# Autodesk Inventor assembly: NSFMRRA10-74-B3-S3-KC31_5-A11(000_000)_MIR_CPY
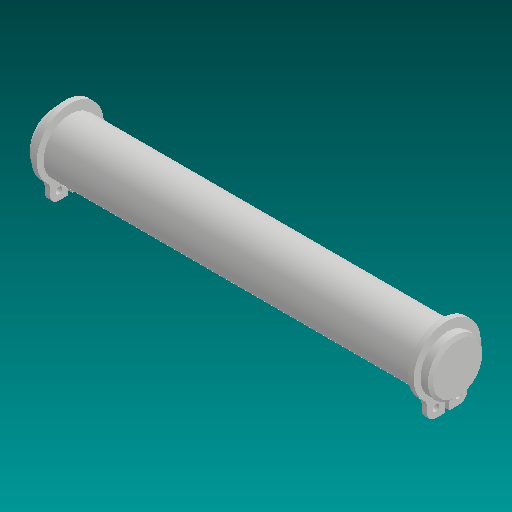
[picture p0: Inventor's stored thumbnail of the model, 512x512]
Saved by Autodesk Inventor 2020 (Build 240168000, 168)
## iProperties
Category: PARTsolutions
Company: MISUMI
Created: 2022-11-16
Part Number: NSFMRRA10-74-B3-S3-KC31_5-A11(000_000)_MIR_CPY
Catalog Web Link: www.cadenas.de
Description: NSFMRR, SFMRR, PSFMRR, SSFMRR, NSFHRR, SFHRR, PSFHRR, SSFHRR, NSFRR, SFRR, PSFRR, SSFRR, NSFMRRA, SFMRRA, PSFMRRA, SSFMRRA, NSFHRRA, SFHRRA, PSFHRRA, SSFHRRA, NSFRRA, SFRRA, PSFRRA, SSFRRA, HFRRA, PHFRRA, PSFRR PSFRRA, PSFHRR, PSFHRRA, SSFRR, SSFRRA, SSFHRR, SSFHRRA, PPSFRR, PPSFRRA, PPSFHRR, PPSFHRRA, SSSFRR, SSSFRRA, SSSFHRR, SSSFHRRA_shaft-Rotary Shafts - Retaining Ring Grooves on Both Ends - Standard
Vendor: MISUMI
Document SubType Name: Assembly
Designer: kanazawakotaro
Manufacturer: MISUMI
Mass: 5.85506 g
Surface Area: 29.329 cm^2
Volume: 5.85506 cm^3
Density: 1 g/cm^3
Title: NSFMRRA10-74-B3-S3-KC31.5-A11
Author: Cadenas PARTsolutions
Comments: Rotary Shafts - Retaining Ring Grooves on Both Ends - Standard
PSOL_IDENT_0: {$CADENAS_DATA/23d-libs/misumi/metric/11_rotary_shafts/psfrra_asmtab.prj},820 {VTYP=3D},{STYP=ASSTAB
PSOL_IDENT_1: },{NB=NSFMRRA10-74-B3-S3-KC31.5-A11(000_000)},{LINA=NSFMRRA10-74-B3-S3-KC31.5-A11},{NN=NSFMRR, SFMRR
PSOL_IDENT_2: , PSFMRR, SSFMRR, NSFHRR, SFHRR, PSFHRR, SSFHRR, NSFRR, SFRR, PSFRR, SSFRR, NSFMRRA, SFMRRA, PSFMRRA
PSOL_IDENT_3: , SSFMRRA, NSFHRRA, SFHRRA, PSFHRRA, SSFHRRA, NSFRRA, SFRRA, PSFRRA, SSFRRA, HFRRA, PHFRRA, PSFRR PS
PSOL_IDENT_4: FRRA, PSFHRR, PSFHRRA, SSFRR, SSFRRA, SSFHRR, SSFHRRA, PPSFRR, PPSFRRA, PPSFHRR, PPSFHRRA, SSSFRR, S
PSOL_IDENT_5: SSFRRA, SSSFHRR, SSSFHRRA_shaft},{DATE=21.04.2022 07:40:19},{GEOMDATE=27.07.2021 08:15:02},{VERSION=
PSOL_IDENT_6: },{LINEID=30},{WBVAR=TS,TYS,MAT,ST,ALT1,L,B,S,ALT2,KC,A,WKC,C,K,E,KZ,Z,ALT3,FC,GALT3,WFC,J,WALT3,V,A
PSOL_IDENT_7: LT4,SFC,SG,AG,ALT5,UC,ALT7,SC,ALT10,KWC,ALT11,WC,ALT32,CD,ALT34,TCJ,WTCJ,XT,HCJ,WHCJ,XH},{WBNUMERIC=
PSOL_IDENT_8: L,B,S,KC,A,WKC,C,K,E,KZ,Z,FC,GALT3,WFC,J,WALT3,V,SFC,SG,AG,UC,SC,KWC,WC,TCJ,WTCJ,XT,HCJ,WHCJ,XH}  {N
PSOL_IDENT_9: B=NSFMRRA10-74-B3-S3-KC31.5-A11(000_000)},{LINA=NSFMRRA10-74-B3-S3-KC31.5-A11},{KT=DUMMY},{PN=NSFMRR
PSOL_IDENT_10: A10-74-B3-S3-KC31.5-A11},{TYPE=NSFMRRA},{TS=SWR},{TYS=H9},{TYSALG= 'H9','h9 (Cold-drawn)','H7','h7 (
PSOL_IDENT_11: Ground)','G6','g6 (Ground)' },{MAT=S45C},{MATALG= 'S45C','S45C Equivalent', 'SUS304','SUS304' },{ST=
PSOL_IDENT_12: },{STALG= '','-','BO','Black Oxide', 'ENP','Electroless Nickel Plating' },{D=10.0},{ALT1=},{ALT1ALG=
PSOL_IDENT_13: '','w/o LKC (Changes L Tolerance)','-LKC','with LKC (Changes L Tolerance)' },{L=74.0},{LALG=[15:800
PSOL_IDENT_14: /0.1]},{LMIN=15},{LMAX=800},{NOTE=25},{B=3.0},{BALG=[3:70/0.1]},{BMAX=70},{S=3.0},{SALG=[3:69/0.1]},
PSOL_IDENT_15: {SMAX=69},{MM=1.15},{DD=9.6},{ARR=STWS10},{ALT2=KC},{ALT2ALG= '', 'w/o Key Grooves','KC','with KC (K
PSOL_IDENT_16: ey Groove)','WKC','with WKC (Two Key Grooves)','KCWKC','with KC + WKC (Three Key Grooves)','KZ','wit
PSOL_IDENT_17: h KC + WKC + KZ (Four Key Grooves)' },{ALT2PN=-KC31.5-A11},{KC=31.5},{KCALG=[0:71/0.1]},{KCMIN=0},{K
PSOL_IDENT_18: CMAX=71},{A=11.0},{AALG=[3:42.5/0.1]},{AMIN=3},{AMAX=42.5},{WKC=0.0},{WKCALG=[0]},{WKCMIN=0},{WKCMAX=
PSOL_IDENT_19: 0},{C=0.0},{CALG=[0]},{CMIN=3},{CMAX=0},{K=0.0},{KALG=[0]},{KMIN=0},{KMAX=69},{E=0.0},{EALG=[0]},{EM
PSOL_IDENT_20: IN=3},{EMAX=72},{KZ=0.0},{KZALG=[0]},{KZMIN=76},{KZMAX=71},{Z=0.0},{ZALG=[0]},{ZMIN=3},{ZMAX=74},{CI
PSOL_IDENT_21: FKC=2},{CIFWKC=1},{CIFK=1},{CIFKZ=2},{PCUT3D=0},{QCUT3D=0},{BB=3},{BBALT2=3},{TT=1.8},{TTALT2=1.8},{
PSOL_IDENT_22: ALT3=},{ALT3ALG= '', 'w/o Set Screw Flat','FC','with FC (Adds a Set Screw Flat)','WFC','with WFC (Ad
PSOL_IDENT_23: ds Two Set Screw Flats)','FCWFC','with FC + WFC (Adds Three Set Screw Flats)' },{ALT3PN=},{FC=0},{FC
PSOL_IDENT_24: ALG=[0]},{FCMIN=0},{FCMAX=73},{GALT3=0},{GALT3ALG=[0]},{GALT3MIN=1},{GALT3MAX=70},{GALT3MAX2=68},{GA
PSOL_IDENT_25: LT3MAX3=70},{WFC=0},{WFCALG=[0]},{WFCMIN=0},{WFCMIN2=2},{WFCMAX=70},{WFCMAX2=-3},{WFCMAX3=-4},{J=0},
PSOL_IDENT_26: {JALG=[0]},{JMIN=1},{JMAX=70},{JMAX2=-2},{JMAX3=-5},{WALT3=0},{WALT3ALG=[0]},{WALT3MIN=0},{WALT3MIN2=
PSOL_IDENT_27: 76},{WALT3MAX=71},{WALT3MAX2=71},{V=0},{VALG=[0]},{VMIN=1},{VMAX=70},{VMAX2=70},{CIFFC=0},{H=0},{ALT
PSOL_IDENT_28: 4=},{ALT4ALG= '', 'w/o SFC (2 Set Screw Flats (Angle Specified))', 'SFC'  , 'with SFC (2 Set Screw F
PSOL_IDENT_29: lats (Angle Specified))'},{ALT4PN=},{SFC=0},{SFCALG=[0]},{SFCMIN=0},{SFCMAX=73},{SG=0},{SGALG=[0]},{
PSOL_IDENT_30: SGMIN=1},{SGMAX=70},{AG=0},{AGALG=[0]},{CIFSFC=0},{ALT5=},{ALT5ALG= '', 'w/o UC (Slit Cam Groove)', '
PSOL_IDENT_31: UC', 'with UC (Slit Cam Groove)'},{ALT5PN=},{UC=0},{UCALG=[0]},{UCMIN=1},{UCMAX=68},{DDALT5=8},{LL1=
PSOL_IDENT_32: 0},{ALT7=},{ALT7ALG= '', 'w/o SC (Wrench Flats)', 'SC', 'with SC (Wrench Flats)'},{ALT7PN=},{SC=0},{
PSOL_IDENT_33: SCALG=[0]},{SCMIN=0},{SCMAX=74},{WALT7=0},{LL2=0},{CIFSC=0},{ALT10=},{ALT10ALG= '','Not applicable'
PSOL_IDENT_34: },{ALT10PN=},{KWC=0},{KWCALG=[0]},{KWCMIN=1},{KWCMAX=0},{WALT10=8},{ALT11=},{ALT11ALG= '','Not appli
PSOL_IDENT_35: cable' },{ALT11PN=},{WC=0.0},{WCALG=[0]},{ALT32=},{ALT32ALG=  '','w/o CD (Changes Part D Chamfering)'
PSOL_IDENT_36: ,'-CD', 'with CD (Changes Part D Chamfering)' },{CD=},{CDALG= '','N/A' },{CD3D=0.5},{CIF32=0},{CIF32
PSOL_IDENT_37: 0=0},{CIF32B=0},{CIF32S=0},{ALT32PN=},{ERRORPN=},{ERRORRALT2=OK},{ERRORRALT3=OK},{ERRORRALT4=NG},{ER
PSOL_IDENT_38: RORRALT5=NG},{ERRORRALT7=NG},{ERRORRALT10=OK},{ERRORALT23=OK},{ERRORALT24=OK},{ERRORALT25=OK},{ERROR
PSOL_IDENT_39: ALT27=OK},{ERRORALT210=OK},{ERRORALT34=OK},{ERRORALT35=OK},{ERRORALT37=OK},{ERRORALT310=OK},{ERRORAL
PSOL_IDENT_40: T45=OK},{ERRORALT47=OK},{ERRORALT410=OK},{ERRORALT75=OK},{ERRORALT510=OK},{ERRORALT710=OK},{ALT34=},
PSOL_IDENT_41: {ALT34ALG= '','Not applicable'},{TCJ=0},{WTCJ=0},{XT=0},{TM=4},{TCJALG=[0]},{TCJMIN=7.000},{TCJMAX=3
PSOL_IDENT_42: 4.000},{TCJMAX1=34.000},{HCJ=0},{WHCJ=0},{XH=0},{HP=4},{HCJALG=[0]},{HCJMIN=7.000},{HCJMAX=34.000},{
PSOL_IDENT_43: HCJMAX1=34.000},{LCJ=0},{LMINX=15},{XALG=[0]},{XCJMIN=7},{PPATH=11_components/psfrra/psfrra_asmtpl.p
PSOL_IDENT_44: rj},{WHCJALG=[0]},{WTCJALG=[0]},{XHALG=[0]}
NB: NSFMRRA10-74-B3-S3-KC31.5-A11(000_000)
NN: NSFMRR, SFMRR, PSFMRR, SSFMRR, NSFHRR, SFHRR, PSFHRR, SSFHRR, NSFRR, SFRR, PSFRR, SSFRR, NSFMRRA, SFMRRA, PSFMRRA, SSFMRRA, NSFHRRA, SFHRRA, PSFHRRA, SSFHRRA, NSFRRA, SFRRA, PSFRRA, SSFRRA, HFRRA, PHFRRA, PSFRR PSFRRA, PSFHRR, PSFHRRA, SSFRR, SSFRRA, SSFHRR, SSFHRRA, PPSFRR, PPSFRRA, PPSFHRR, PPSFHRRA, SSSFRR, SSSFRRA, SSSFHRR, SSSFHRRA_shaft
NT: Rotary Shafts - Retaining Ring Grooves on Both Ends - Standard
NBSYN: $PN.($ALT34.$TCJ.$WTCJ.$XT._$HCJ.$WHCJ.$XH.)
LINA: NSFMRRA10-74-B3-S3-KC31.5-A11
CATALOG: Misumi
PN: NSFMRRA10-74-B3-S3-KC31.5-A11
TS: With Retaining Ring
TYS: h9 (Cold-drawn)
MAT: S45C Equivalent
ST: -
D: 10
ALT1: w/o LKC (Changes L Tolerance)
L: 74
B: 3
S: 3
MM: 1.15
DD: 9.6
ALT2: with KC (Key Groove)
KC: 31.5
A: 11
WKC: 0
C: 0
K: 0
E: 0
KZ: 0
Z: 0
ALT3: w/o Set Screw Flat
FC: 0
GALT3: 0
WFC: 0
J: 0
WALT3: 0
V: 0
ALT4: w/o SFC (2 Set Screw Flats (Angle Specified))
SFC: 0
SG: 0
AG: 0
ALT5: w/o UC (Slit Cam Groove)
UC: 0
ALT7: w/o SC (Wrench Flats)
SC: 0
ALT10: Not applicable
KWC: 0
ALT11: Not applicable
WC: 0
ALT32: w/o CD (Changes Part D Chamfering)
CD: N/A
ALT34: Not applicable
TCJ: 0
WTCJ: 0
XT: 0
HCJ: 0
WHCJ: 0
XH: 0
SUPPLIER: MISUMI
ARTICLENO: NSFMRRA10-74-B3-S3-KC31.5-A11(000_000)
BOMINFO: NSFMRRA10-74-B3-S3-KC31.5-A11
CREATOR: CADENAS GmbH
## Documents named in this file (3)
- C:\Users\金澤航太郎\Documents\Inventor\kamuy2\Parts\NSFMRRA10-74-B3-S3-KC31.5-A11_Autodesk_Inventor_2020_20221116\AIS2020\NSFMRRA10-74-B3-S3-KC31_5-A11(000_000)_MIR_CPY.iam
- C:\Users\金澤航太郎\Documents\Inventor\kamuy2\Parts\NSFMRRA10-74-B3-S3-KC31.5-A11_Autodesk_Inventor_2020_20221116\AIS2020\NSFMRRA10-74-B3-S3-KC31_5-A11(000_000)_s_MIR_CPY.ipt
- C:\Users\金澤航太郎\Documents\Inventor\kamuy2\Parts\NSFMRRA10-74-B3-S3-KC31.5-A11_Autodesk_Inventor_2020_20221116\AIS2020\STWN10_MIR_CPY.ipt
## Components (3 placed, 2 different names)
1. NSFMRRA10-74-B3-S3-KC31_5-A11(000_000)_s_MIR_CPY:1 — to_ring_b_XY@1 <-> 1_XY@2, to_ring_b_Z@1 <-> 1_Z@2, to_ring_s_XY@1 <-> 1_XY@3, to_ring_s_Z@1 <-> 1_Z@3, to_ring_b_YZ@1 <-> 1_YZ@2, to_ring_s_YZ@1 <-> 1_YZ@3
2. STWN10_MIR_CPY:1 — to_ring_b_XY@1 <-> 1_XY@2, to_ring_b_Z@1 <-> 1_Z@2, to_ring_b_YZ@1 <-> 1_YZ@2
3. STWN10_MIR_CPY:2 — to_ring_s_XY@1 <-> 1_XY@3, to_ring_s_Z@1 <-> 1_Z@3, to_ring_s_YZ@1 <-> 1_YZ@3
## Relationships (6: Mate 3, Angle 2, Flush 1)
- to_ring_b_XY@1 <-> 1_XY@2 [Mate]: NSFMRRA10-74-B3-S3-KC31_5-A11(000_000)_s_MIR_CPY:1 ↔ STWN10_MIR_CPY:1
- to_ring_b_Z@1 <-> 1_Z@2 [Mate]: NSFMRRA10-74-B3-S3-KC31_5-A11(000_000)_s_MIR_CPY:1 ↔ STWN10_MIR_CPY:1
- to_ring_s_XY@1 <-> 1_XY@3 [Flush]: NSFMRRA10-74-B3-S3-KC31_5-A11(000_000)_s_MIR_CPY:1 ↔ STWN10_MIR_CPY:2
- to_ring_s_Z@1 <-> 1_Z@3 [Mate]: NSFMRRA10-74-B3-S3-KC31_5-A11(000_000)_s_MIR_CPY:1 ↔ STWN10_MIR_CPY:2
- to_ring_b_YZ@1 <-> 1_YZ@2 [Angle] (-180 deg): NSFMRRA10-74-B3-S3-KC31_5-A11(000_000)_s_MIR_CPY:1 ↔ STWN10_MIR_CPY:1
- to_ring_s_YZ@1 <-> 1_YZ@3 [Angle] (0 deg): NSFMRRA10-74-B3-S3-KC31_5-A11(000_000)_s_MIR_CPY:1 ↔ STWN10_MIR_CPY:2
